# Autodesk Inventor assembly: Сборка_Конечная
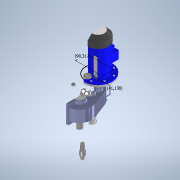
[picture p0: Inventor's stored thumbnail of the model, 180x180]
Saved by Autodesk Inventor 2021 (Build 250183000, 183)
## iProperties
Created: 2023-04-17
Part Number: Сборка_Конечная
Document SubType Name: Assembly
Designer: gdevc
Mass: 20498.7 g
Surface Area: 13360.1 cm^2
Volume: 12308.6 cm^3
Density: 1.66539 g/cm^3
Author: gdevc
## Documents named in this file (18)
- C:\Users\gdevc\OneDrive\Рабочий стол\Курсач\DetaliMashine\Новая папка\Сборка_Конечная.iam
- C:\Users\gdevc\OneDrive\Рабочий стол\Курсач\DetaliMashine\Новая папка\Корпус.v.2.0.iam
- C:\Users\gdevc\OneDrive\Рабочий стол\Курсач\DetaliMashine\Новая папка\Вал_тихоходный.ipt
- C:\Users\gdevc\OneDrive\Рабочий стол\Курсач\DetaliMashine\Новая папка\Вал_промежуточный.ipt
- C:\Users\gdevc\OneDrive\Рабочий стол\Курсач\DetaliMashine\Новая папка\Валл быстроходный.ipt
- C:\Users\gdevc\OneDrive\Рабочий стол\Курсач\DetaliMashine\Новая папка\Крышка, тихая.ipt
- C:\Users\gdevc\OneDrive\Рабочий стол\Курсач\DetaliMashine\Новая папка\Крышка тих_выход.ipt
- C:\Users\gdevc\OneDrive\Рабочий стол\Курсач\DetaliMashine\Новая папка\Крышка_пром.ipt
- C:\Users\gdevc\OneDrive\Рабочий стол\Курсач\DetaliMashine\Новая папка\Подшипник 210 ГОСТ 8338-75.ipt
- C:\Users\gdevc\OneDrive\Рабочий стол\Курсач\DetaliMashine\Новая папка\Колесо быстроходное.ipt
- C:\Users\gdevc\OneDrive\Рабочий стол\Курсач\DetaliMashine\Новая папка\Манжет 2-50x65x8 ГОСТ 8752-79.ipt
- C:\Users\gdevc\OneDrive\Рабочий стол\Курсач\DetaliMashine\Новая папка\Манжет 1-30x47x7 ГОСТ 8752-79.ipt
- C:\Users\gdevc\OneDrive\Рабочий стол\Курсач\DetaliMashine\Новая папка\Крышка_быстроходного.ipt
- C:\Users\gdevc\OneDrive\Рабочий стол\Курсач\DetaliMashine\Новая папка\Промежуточное колесо резина.ipt
- C:\Users\gdevc\OneDrive\Рабочий стол\Курсач\DetaliMashine\Новая папка\Резина конец.ipt
- C:\Users\gdevc\Downloads\Telegram Desktop\АИР100L IM2081 (2,4,6,8 пол)....ipt
- C:\Users\gdevc\OneDrive\Документы\Inventor\Content Center Files\R2021\ru-RU\GOST 5915-70\Гайка M16-6H ГОСТ 5915-70(1).ipt
- C:\Users\gdevc\OneDrive\Рабочий стол\Курсач\DetaliMashine\Новая папка\Подшипник 7205A ГОСТ 27365-8v.1.ipt
## Components (20 placed, 17 different names)
1. Корпус.v.2.0:1 [sub-assembly]
2. Вал_тихоходный:1 — Совмещение:1, Угол:6
3. Вал_промежуточный:1
4. Валл быстроходный:1 — Угол:1, Совмещение:35, Совмещение:37
5. Крышка, тихая:1
6. Крышка тих_выход:1
7. Крышка_пром:1
8. Крышка_пром:2
9. Подшипник 210 ГОСТ 8338-75:1
10. Подшипник 210 ГОСТ 8338-75:2
11. Колесо быстроходное:1
12. Манжет 2-50x65x8 ГОСТ 8752-79:1
13. Манжет 1-30x47x7 ГОСТ 8752-79:1
14. Крышка_быстроходного:1
15. Промежуточное колесо резина:1
16. Резина конец:1
17. АИР100L IM2081 (2,4,6,8 пол)...:1
18. Гайка ГОСТ 5915-70 M16:1 — Совмещение:35, Совмещение:37
19. Подшипник 7205A ГОСТ 27365-8v.1:1
20. Подшипник 7205A ГОСТ 27365-8v.1:2
## Relationships (5: Mate 3, Angle 2)
- Совмещение:1 [Mate]: Вал_тихоходный:1
- Угол:1 [Angle] (0 deg): Валл быстроходный:1
- Совмещение:35 [Mate] (107.5 mm): Валл быстроходный:1 ↔ Гайка ГОСТ 5915-70 M16:1
- Совмещение:37 [Mate] (215 mm): Валл быстроходный:1 ↔ Гайка ГОСТ 5915-70 M16:1
- Угол:6 [Angle] (180 deg): Вал_тихоходный:1
